# Autodesk Inventor assembly: MainBody
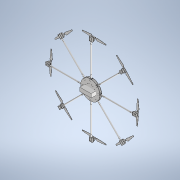
[picture p0: Inventor's stored thumbnail of the model, 180x180]
Saved by Autodesk Inventor 2022.1 (Build 261234020, 234B)
## iProperties
Created: 2021-11-14
Part Number: MainBody
Document SubType Name: Assembly
Designer: Alexander
Author: Alexander
## Documents named in this file (5)
- C:\Users\Alexander\Desktop\upload\Drone\3D models\MainBody.iam
- C:\Users\Alexander\Desktop\upload\Drone\3D models\Arm.iam
- C:\Users\Alexander\Desktop\upload\Drone\3D models\MainDisk1.ipt
- C:\Users\Alexander\Desktop\upload\Drone\3D models\ESC.ipt
- C:\Users\Alexander\Desktop\upload\Drone\3D models\Battery.ipt
## Components (19 placed, 4 different names)
1. MainDisk1:1 — Mate:9, Rigid:1
2. MainDisk1:2 — Mate:10, Mate:11, Mate:12
3. Battery:1 — Rigid:1
4. ESC:1
5. ESC:2
6. ESC:3
7. ESC:4
8. ESC:5
9. ESC:6
10. ESC:7
11. ESC:8
12. Arm:1 [sub-assembly] — Mate:9, Mate:10, Mate:11, Mate:12
13. Arm:2 [sub-assembly]
14. Arm:3 [sub-assembly]
15. Arm:4 [sub-assembly]
16. Arm:5 [sub-assembly]
17. Arm:6 [sub-assembly]
18. Arm:7 [sub-assembly]
19. Arm:8 [sub-assembly]
## Component patterns: (8 elements, first: ESC:1), (8 elements, first: Arm:1)
## Relationships (5: Mate 4, WeldJoint 1)
- Mate:9: MainDisk1:1 ↔ Arm:1
- Mate:10: MainDisk1:2 ↔ Arm:1
- Mate:11: MainDisk1:2 ↔ Arm:1
- Mate:12: MainDisk1:2 ↔ Arm:1
- Rigid:1 [WeldJoint]: MainDisk1:1 ↔ Battery:1
